# Autodesk Inventor assembly: Ensemble voir si c'est plat
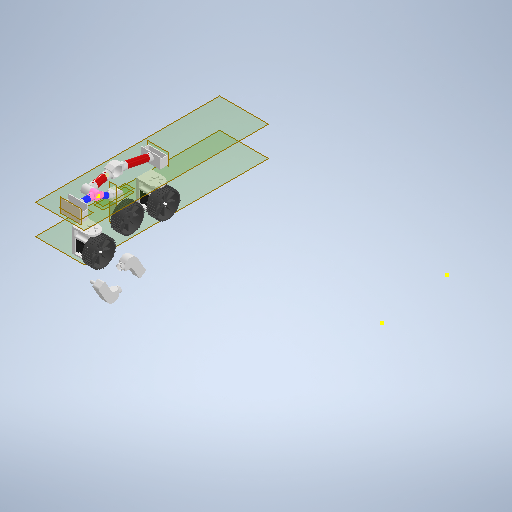
[picture p0: Inventor's stored thumbnail of the model, 512x512]
Saved by Autodesk Inventor 2026.2 (Build 302298010, 298A)
## iProperties
Created: 2026-05-12
Part Number: Ensemble voir si c'est plat
Document SubType Name: Assembly
Designer: Genon
Author: Genon
## Documents named in this file (15)
- C:\Users\genon\Documents\Henallux Passerelle\Projet de conception\Cassini T-X\Inventor\Ensemble voir si c'est plat.iam
- C:\Users\genon\Documents\Henallux Passerelle\Projet de conception\Cassini T-X\Inventor\Suspension\bielle côté 3.ipt
- C:\Users\genon\Documents\Henallux Passerelle\Projet de conception\Cassini T-X\Inventor\Suspension\tube vers bogie.ipt
- C:\Users\genon\Documents\Henallux Passerelle\Projet de conception\Cassini T-X\Inventor\Suspension\tubelong_rocker.ipt
- C:\Users\genon\Documents\Henallux Passerelle\Projet de conception\Cassini T-X\Inventor\Suspension\Attache servomoteur.ipt
- C:\Users\genon\Documents\Henallux Passerelle\Projet de conception\Cassini T-X\Inventor\Suspension\Attache servomoteur_bogie.ipt
- C:\Users\genon\Documents\Henallux Passerelle\Projet de conception\Cassini T-X\Inventor\Suspension\bielle rocker.ipt
- C:\Users\genon\Documents\Henallux Passerelle\Projet de conception\Cassini T-X\Inventor\Suspension\bielle rocker2.ipt
- C:\Users\genon\Documents\Henallux Passerelle\Projet de conception\Cassini T-X\Inventor\Suspension\tube des bogies.ipt
- C:\Users\genon\Documents\Henallux Passerelle\Projet de conception\Cassini T-X\Inventor\Suspension\support palonnier test.ipt
- C:\Users\genon\Documents\Henallux Passerelle\Projet de conception\Cassini T-X\Inventor\Composants\Stepper Motor\Stepper Motor\Stepper Motor.ipt
- C:\Users\genon\Documents\Henallux Passerelle\Projet de conception\Cassini T-X\Inventor\Suspension\Roue.ipt
- C:\Users\genon\Documents\Henallux Passerelle\Projet de conception\Cassini T-X\Inventor\Suspension\Roue libre.ipt
- C:\Users\genon\Documents\Henallux Passerelle\Projet de conception\Cassini T-X\Inventor\Suspension\bielle roue milieu autre côté.ipt
- C:\Users\genon\Documents\Henallux Passerelle\Projet de conception\Cassini T-X\Inventor\Suspension\bielle roue milieu autre .ipt
## Components (19 placed, 14 different names)
1. bielle côté 3:1 — Placage:1, Placage:2, Placage:3, Placage:4, Placage:5, Placage:6
2. tube vers bogie:2 — Placage:1, Placage:2, Placage:3, Placage:7, Placage:8, Placage:9
3. tubelong_rocker:2 — Placage:4, Placage:5, Placage:6, Placage:10, Placage:11, Placage:12
4. Attache servomoteur:3 — Placage:10, Placage:11, Placage:12, Affleurement:1, Placage:25, Affleurement:8
5. Attache servomoteur_bogie:1 — Placage:21, Placage:22, Placage:23, Affleurement:2, Placage:24, Affleurement:6
6. bielle rocker:2 — Placage:7, Placage:8, Placage:9, Placage:13, Placage:14
7. bielle rocker2:1 — Placage:13, Placage:14, Placage:15, Placage:16, Placage:17, Placage:18, Placage:19, Placage:20
8. tube des bogies:1 — Placage:15, Placage:16, Placage:17, Placage:21, Placage:22, Placage:23
9. tube des bogies:2 — Placage:18, Placage:19, Placage:20, Placage:36, Placage:37, Placage:38
10. support palonnier test:2 — Placage:24, Placage:26, Affleurement:5, Placage:29, Placage:30, Affleurement:7
11. support palonnier test:3 — Placage:25, Placage:32, Affleurement:9, Affleurement:10, Placage:34, Placage:35
12. Stepper Motor:2 — Placage:26, Affleurement:5, Placage:29, Placage:31
13. Stepper Motor:3 — Placage:33, Affleurement:10, Placage:34, Placage:35
14. Roue:1 — Placage:30, Placage:31
15. Roue:2 — Placage:32, Placage:33
16. Roue libre:1 — Placage:39
17. bielle roue milieu autre côté:2 — Placage:36, Placage:37, Placage:38, Placage:39
18. bielle roue milieu autre :1
19. bielle roue milieu autre :2
## Relationships (49: Mate 37, Flush 9, Angle 3)
- Placage:1 [Mate]: bielle côté 3:1 ↔ tube vers bogie:2
- Placage:2 [Mate]: bielle côté 3:1 ↔ tube vers bogie:2
- Placage:3 [Mate]: bielle côté 3:1 ↔ tube vers bogie:2
- Placage:4 [Mate]: bielle côté 3:1 ↔ tubelong_rocker:2
- Placage:5 [Mate]: bielle côté 3:1 ↔ tubelong_rocker:2
- Placage:6 [Mate]: bielle côté 3:1 ↔ tubelong_rocker:2
- Placage:7 [Mate]: tube vers bogie:2 ↔ bielle rocker:2
- Placage:8 [Mate]: tube vers bogie:2 ↔ bielle rocker:2
- Placage:9 [Mate]: tube vers bogie:2 ↔ bielle rocker:2
- Placage:10 [Mate]: tubelong_rocker:2 ↔ Attache servomoteur:3
- Placage:11 [Mate]: tubelong_rocker:2 ↔ Attache servomoteur:3
- Placage:12 [Mate]: tubelong_rocker:2 ↔ Attache servomoteur:3
- Placage:13 [Mate]: bielle rocker:2 ↔ bielle rocker2:1
- Placage:14 [Mate]: bielle rocker:2 ↔ bielle rocker2:1
- Placage:15 [Mate]: bielle rocker2:1 ↔ tube des bogies:1
- Placage:16 [Mate]: bielle rocker2:1 ↔ tube des bogies:1
- Placage:17 [Mate]: bielle rocker2:1 ↔ tube des bogies:1
- Placage:18 [Mate]: bielle rocker2:1 ↔ tube des bogies:2
- Placage:19 [Mate]: bielle rocker2:1 ↔ tube des bogies:2
- Placage:20 [Mate]: bielle rocker2:1 ↔ tube des bogies:2
- Placage:21 [Mate]: Attache servomoteur_bogie:1 ↔ tube des bogies:1
- Placage:22 [Mate]: Attache servomoteur_bogie:1 ↔ tube des bogies:1
- Placage:23 [Mate]: Attache servomoteur_bogie:1 ↔ tube des bogies:1
- Affleurement:1 [Flush]: Attache servomoteur:3
- Affleurement:2 [Flush]: Attache servomoteur_bogie:1
- Angle:1 (0 deg)
- Placage:24 [Mate] (4.3 mm): Attache servomoteur_bogie:1 ↔ support palonnier test:2
- Placage:25 [Mate] (4.3 mm): Attache servomoteur:3 ↔ support palonnier test:3
- Placage:26 [Mate]: support palonnier test:2 ↔ Stepper Motor:2
- Affleurement:5 [Flush] (2 mm): support palonnier test:2 ↔ Stepper Motor:2
- Placage:29 [Mate]: support palonnier test:2 ↔ Stepper Motor:2
- Placage:30 [Mate]: support palonnier test:2 ↔ Roue:1
- Placage:31 [Mate]: Stepper Motor:2 ↔ Roue:1
- Placage:32 [Mate]: support palonnier test:3 ↔ Roue:2
- Placage:33 [Mate]: Stepper Motor:3 ↔ Roue:2
- Affleurement:6 [Flush]: Attache servomoteur_bogie:1
- Affleurement:7 [Flush]: support palonnier test:2
- Angle:2 (0 deg)
- Affleurement:8 [Flush]: Attache servomoteur:3
- Affleurement:9 [Flush]: support palonnier test:3
- Angle:3 (0 deg)
- Affleurement:10 [Flush] (2 mm): support palonnier test:3 ↔ Stepper Motor:3
- Placage:34 [Mate]: support palonnier test:3 ↔ Stepper Motor:3
- Placage:35 [Mate]: support palonnier test:3 ↔ Stepper Motor:3
- Placage:36 [Mate]: tube des bogies:2 ↔ bielle roue milieu autre côté:2
- Placage:37 [Mate]: tube des bogies:2 ↔ bielle roue milieu autre côté:2
- Placage:38 [Mate]: tube des bogies:2 ↔ bielle roue milieu autre côté:2
- Affleurement:11 [Flush] (94.05 mm)
- Placage:39 [Mate]: Roue libre:1 ↔ bielle roue milieu autre côté:2
